# Autodesk Inventor assembly: ScannerSetUp
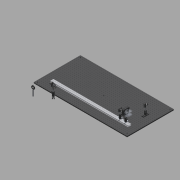
[picture p0: Inventor's stored thumbnail of the model, 180x180]
Saved by Autodesk Inventor 2018 (Build 220112000, 112)
## iProperties
Created: 2018-09-17
Part Number: ScannerSetUp
Document SubType Name: Assembly
Designer: Robert Campbell
Author: Robert Campbell
## Documents named in this file (8)
- X:\home\work\Documents\MF_BenchOptics\CAD_files\ScannerSetUp.iam
- X:\home\work\Documents\MF_BenchOptics\CAD_files\MB60120_M-Solidworks.ipt
- X:\home\work\Documents\MF_BenchOptics\CAD_files\XT66DP-1000-Solidworks.ipt
- X:\home\work\Documents\MF_BenchOptics\CAD_files\first_mirror.iam
- X:\home\work\Documents\MF_BenchOptics\CAD_files\MountedScanners.iam
- W:\home\work\Documents\MF_BenchOptics\CAD_files\SM1_scanlensholder_on_mount.iam
- W:\home\work\Documents\MF_BenchOptics\CAD_files\ID25_M-Solidworks.ipt
- W:\home\work\Documents\MF_BenchOptics\CAD_files\first_mirror.iam
## Components (7 placed, 6 different names)
1. MB60120_M-Solidworks:1 — Mate:1, Mate:21
2. XT66DP-1000-Solidworks:1 — Mate:1, Angle:1, Mate:22, Mate:29
3. first_mirror:1 [sub-assembly] — Mate:21
4. MountedScanners:1 [sub-assembly] — Angle:1, Mate:22
5. SM1_scanlensholder_on_mount:1 [sub-assembly] — Mate:29
6. ID25_M-Solidworks:1
7. first_mirror:2 [sub-assembly]
## Relationships (5: Mate 4, Angle 1)
- Mate:1: MB60120_M-Solidworks:1 ↔ XT66DP-1000-Solidworks:1
- Mate:21: MB60120_M-Solidworks:1 ↔ first_mirror:1
- Angle:1 (0 deg): XT66DP-1000-Solidworks:1 ↔ MountedScanners:1
- Mate:22: XT66DP-1000-Solidworks:1 ↔ MountedScanners:1
- Mate:29: XT66DP-1000-Solidworks:1 ↔ SM1_scanlensholder_on_mount:1
